# Autodesk Inventor assembly: montagem
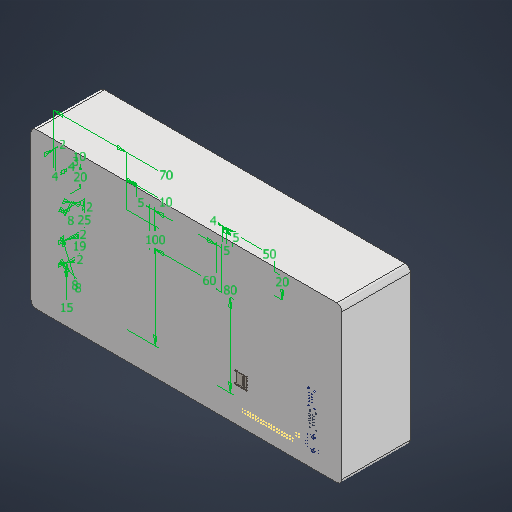
[picture p0: Inventor's stored thumbnail of the model, 512x512]
Saved by Autodesk Inventor 2027 (Build 310192060, 192F)
## iProperties
Created: 2026-04-26
Part Number: montagem
Document SubType Name: Assembly
Designer: Lucas David
Author: Lucas David
## Documents named in this file (9)
- C:\Users\Visitante\Downloads\IC (1)-20260628T134607Z-3-001\IC (1)\montagem (1).iam
- C:\Users\Visitante\Downloads\jehan.ipt
- C:\Users\Visitante\Downloads\IC (1)-20260628T134607Z-3-001\IC (1)\Transmissor (1).ipt
- C:\Users\Visitante\Downloads\IC (1)-20260628T134607Z-3-001\IC (1)\receptor ftth fibra (1).ipt
- C:\Users\Visitante\Downloads\IC (1)-20260628T134607Z-3-001\IC (1)\Repetidor (1).ipt
- C:\Users\Visitante\Downloads\IC (1)-20260628T134607Z-3-001\IC (1)\bateria (1).ipt
- C:\Users\Lucas David\Downloads\raspberry_pi_5\raspberry_pi_5\raspberry_pi_5.iam
- C:\Users\Visitante\Downloads\IC (1)-20260628T134607Z-3-001\IC (1)\transdutor (1).ipt
- C:\Users\Visitante\Downloads\Ic.jehan-20260627T111651Z-3-001\Ic.jehan\Raspberry Pi 4 Model B\Raspberry Pi 4 Model B.iam
## Components (8 placed, 8 different names)
1. jehan:1 — Coincidente:1, Rígida:1, Coincidente:2, Coincidente:3, Coincidente:4, Coincidente:5, Coincidente:6, Coincidente:7, Coincidente:8, Coincidente:9, Coincidente:10, Coincidente:11, Coincidente:12, Coincidente:13, Alinhado:1, Coincidente:14, Coincidente:15, Coincidente:16
2. Transmissor (1):1 — Coincidente:1, Coincidente:2, Coincidente:3, Coincidente:4, Coincidente:5
3. receptor ftth fibra (1):1 — Coincidente:8, Coincidente:9
4. Repetidor (1):1 — Coincidente:6, Coincidente:7
5. bateria (1):1 — Coincidente:10, Coincidente:11, Coincidente:12
6. raspberry_pi_5:1 [sub-assembly] — Rígida:1
7. transdutor (1):1 — Coincidente:13, Alinhado:1, Coincidente:15, Coincidente:16
8. Raspberry Pi 4 Model B:1 [sub-assembly] — Coincidente:14
## Relationships (18: Mate 16, WeldJoint 1, Flush 1)
- Coincidente:1 [Mate]: jehan:1 ↔ Transmissor (1):1
- Rígida:1 [WeldJoint]: jehan:1 ↔ raspberry_pi_5:1
- Coincidente:2 [Mate]: jehan:1 ↔ Transmissor (1):1
- Coincidente:3 [Mate]: jehan:1 ↔ Transmissor (1):1
- Coincidente:4 [Mate] (7.5 mm): jehan:1 ↔ Transmissor (1):1
- Coincidente:5 [Mate] (3 mm): jehan:1 ↔ Transmissor (1):1
- Coincidente:6 [Mate]: jehan:1 ↔ Repetidor (1):1
- Coincidente:7 [Mate] (3 mm): jehan:1 ↔ Repetidor (1):1
- Coincidente:8 [Mate]: jehan:1 ↔ receptor ftth fibra (1):1
- Coincidente:9 [Mate] (3 mm): jehan:1 ↔ receptor ftth fibra (1):1
- Coincidente:10 [Mate]: jehan:1 ↔ bateria (1):1
- Coincidente:11 [Mate] (10 mm): jehan:1 ↔ bateria (1):1
- Coincidente:12 [Mate] (15 mm): jehan:1 ↔ bateria (1):1
- Coincidente:13 [Mate]: jehan:1 ↔ transdutor (1):1
- Alinhado:1 [Flush] (65 mm): jehan:1 ↔ transdutor (1):1
- Coincidente:14 [Mate]: jehan:1 ↔ Raspberry Pi 4 Model B:1
- Coincidente:15 [Mate]: jehan:1 ↔ transdutor (1):1
- Coincidente:16 [Mate] (125 mm): jehan:1 ↔ transdutor (1):1
